# Autodesk Inventor assembly: Solenoid
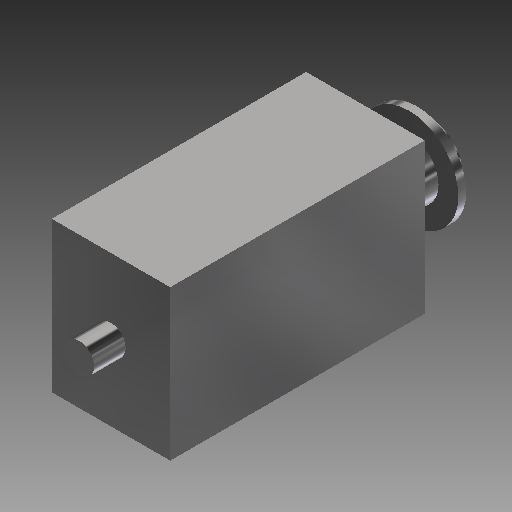
[picture p0: Inventor's stored thumbnail of the model, 512x512]
Saved by Autodesk Inventor 2019 (Build 230136000, 136)
## iProperties
Created: 2018-11-02
Part Number: Solenoid
Document SubType Name: Assembly
Designer: Ethan
Author: Ethan
## Documents named in this file (3)
- C:\Users\Ethan\Documents\SE101\3D Models\Solenoid.iam
- C:\Users\Ethan\Documents\SE101\3D Models\Solenoid Body.ipt
- C:\Users\Ethan\Documents\SE101\3D Models\Solenoid Arm.ipt
## Components (2 placed, 2 different names)
1. Solenoid Body:1 — Cylindrical:1
2. Solenoid Arm:1 — Cylindrical:1
## Relationships (1: CylindricalJoint 1)
- Cylindrical:1: Solenoid Body:1 ↔ Solenoid Arm:1
